# Autodesk Inventor assembly: ASY Beshkino_bio_tank_work
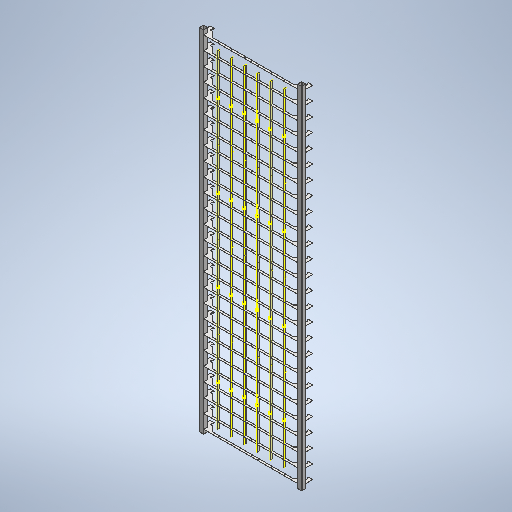
[picture p0: Inventor's stored thumbnail of the model, 512x512]
Saved by Autodesk Inventor 2025 (Build 290162010, 162A)
## iProperties
Created: 2024-07-23
Part Number: ASY Beshkino_bio_tank_work
Document SubType Name: Assembly
Designer: pokla
Author: pokla
## Documents named in this file (4)
- C:\Users\pokla\Documents\Inventor\BSH_Beshkino_bio_tank\ASY Beshkino_bio_tank_work.iam
- C:\Users\pokla\Documents\Inventor\BSH_Beshkino_bio_tank\BSH 021 rib 1.ipt
- C:\Users\pokla\Documents\Inventor\BSH_Beshkino_bio_tank\BSH 061 tube 1.ipt
- C:\Users\pokla\Documents\Inventor\BSH_Beshkino_bio_tank\BSH 041 stringer floor.ipt
## Components (78 placed, 3 different names)
1. BSH 061 tube 1:1 — Mate:1, Mate:2, Flush:1, Rigid:2, Flush:2, Mate:3, Mate:4
2. BSH 061 tube 1:2 — Rigid:2
3. BSH 020 rib 1:2 — Rigid:1, Flush:2, Mate:3, Mate:4
4. BSH 020 rib 1:1 — Rigid:1
5. BSH 020 rib 1:3
6. BSH 020 rib 1:4 — Rigid:3
7. BSH 020 rib 1:5
8. BSH 020 rib 1:6
9. BSH 020 rib 1:7
10. BSH 020 rib 1:8
11. BSH 020 rib 1:9
12. BSH 020 rib 1:10
13. BSH 020 rib 1:11
14. BSH 020 rib 1:12
15. BSH 020 rib 1:13
16. BSH 020 rib 1:14
17. BSH 020 rib 1:15
18. BSH 020 rib 1:16
19. BSH 020 rib 1:17
20. BSH 020 rib 1:18
21. BSH 020 rib 1:19
22. BSH 020 rib 1:20
23. BSH 020 rib 1:21
24. BSH 020 rib 1:22
25. BSH 020 rib 1:23
26. BSH 020 rib 1:24
27. BSH 020 rib 1:25
28. BSH 020 rib 1:26
29. BSH 020 rib 1:27
30. BSH 020 rib 1:28
31. BSH 020 rib 1:29
32. BSH 020 rib 1:30
33. BSH 020 rib 1:31
34. BSH 020 rib 1:32
35. BSH 020 rib 1:33
36. BSH 020 rib 1:34
37. BSH 020 rib 1:35
38. BSH 020 rib 1:36
39. BSH 020 rib 1:37
40. BSH 020 rib 1:38
41. BSH 020 rib 1:39
42. BSH 020 rib 1:40
43. BSH 020 rib 1:41
44. BSH 020 rib 1:42
45. BSH 020 rib 1:43
46. BSH 020 rib 1:44
47. BSH 020 rib 1:45
48. BSH 020 rib 1:46
49. BSH 020 rib 1:47
50. BSH 020 rib 1:48
51. BSH 020 rib 1:49
52. BSH 020 rib 1:50
53. BSH 020 rib 1:51
54. BSH 020 rib 1:52
55. BSH 041 stringer floor:1 — Rigid:3, Rigid:4
56. BSH 041 stringer floor:2 — Rigid:4, Rigid:6
57. BSH 041 stringer floor:3 — Rigid:6
58. BSH 041 stringer floor:4
59. BSH 041 stringer floor:5
60. BSH 041 stringer floor:6
61. BSH 041 stringer floor:7
62. BSH 041 stringer floor:8
63. BSH 041 stringer floor:9
64. BSH 041 stringer floor:10
65. BSH 041 stringer floor:11
66. BSH 041 stringer floor:12
67. BSH 041 stringer floor:13
68. BSH 041 stringer floor:14
69. BSH 041 stringer floor:15
70. BSH 041 stringer floor:16
71. BSH 041 stringer floor:17
72. BSH 041 stringer floor:18
73. BSH 041 stringer floor:19
74. BSH 041 stringer floor:20
75. BSH 041 stringer floor:21
76. BSH 041 stringer floor:22
77. BSH 041 stringer floor:23
78. BSH 041 stringer floor:24
## Component patterns: (26 elements, first: BSH 020 rib 1:2 + BSH 020 rib 1:1), (6 elements, first: BSH 041 stringer floor:1 + BSH 041 stringer floor:2 + BSH 041 stringer floor:3 + BSH 041 stringer floor:4)
## Relationships (12: WeldJoint 6, Mate 4, Flush 2)
- Rigid:1 [WeldJoint]: BSH 020 rib 1:2 ↔ BSH 020 rib 1:1
- Mate:1: BSH 061 tube 1:1
- Mate:2 (2300 mm): BSH 061 tube 1:1
- Flush:1: BSH 061 tube 1:1
- Rigid:2 [WeldJoint] (2200 mm): BSH 061 tube 1:1 ↔ BSH 061 tube 1:2
- Flush:2 (100 mm): BSH 061 tube 1:1 ↔ BSH 020 rib 1:2
- Mate:3: BSH 061 tube 1:1 ↔ BSH 020 rib 1:2
- Mate:4: BSH 061 tube 1:1 ↔ BSH 020 rib 1:2
- Rigid:3 [WeldJoint] (2 mm): BSH 020 rib 1:4 ↔ BSH 041 stringer floor:1
- Rigid:4 [WeldJoint]: BSH 041 stringer floor:1 ↔ BSH 041 stringer floor:2
- [WeldJoint]: BSH 041 stringer floor:3 ↔ BSH 041 stringer floor:4
- Rigid:6 [WeldJoint]: BSH 041 stringer floor:2 ↔ BSH 041 stringer floor:3
## Named parameters: d21_d20 = 0 mm
